# Autodesk Inventor assembly: Layout
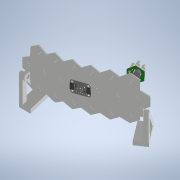
[picture p0: Inventor's stored thumbnail of the model, 180x180]
Saved by Autodesk Inventor 2022.1 (Build 261234020, 234B)
## iProperties
Created: 2021-11-18
Part Number: Layout
Document SubType Name: Assembly
Designer: Eric
Author: Eric
## Documents named in this file (5)
- C:\repo\IRheating\3dModels\Layout.iam
- C:\repo\IRheating\KiCAD\sevenLEDboard.ipt
- C:\repo\IRheating\3dModels\ArrayBracket.ipt
- C:\repo\IRheating\3dModels\Camara_MLX90640.ipt
- C:\repo\IRheating\3dModels\ArrayBracketSupport.ipt
## Components (5 placed, 4 different names)
1. sevenLEDboard:1 — Mate:1, Angle:1, Mate:2
2. ArrayBracket:1 — Mate:1, Angle:1, Mate:2, Insert:2, Insert:3, Insert:4
3. Camara_MLX90640:1 — Insert:2
4. ArrayBracketSupport:1 — Insert:3
5. ArrayBracketSupport:2 — Insert:4
## Relationships (6: Insert 3, Mate 2, Angle 1)
- Mate:1: sevenLEDboard:1 ↔ ArrayBracket:1
- Angle:1 (0 deg): sevenLEDboard:1 ↔ ArrayBracket:1
- Mate:2: sevenLEDboard:1 ↔ ArrayBracket:1
- Insert:2: ArrayBracket:1 ↔ Camara_MLX90640:1
- Insert:3: ArrayBracket:1 ↔ ArrayBracketSupport:1
- Insert:4: ArrayBracket:1 ↔ ArrayBracketSupport:2
